# Autodesk Inventor assembly: 6P Sprocket
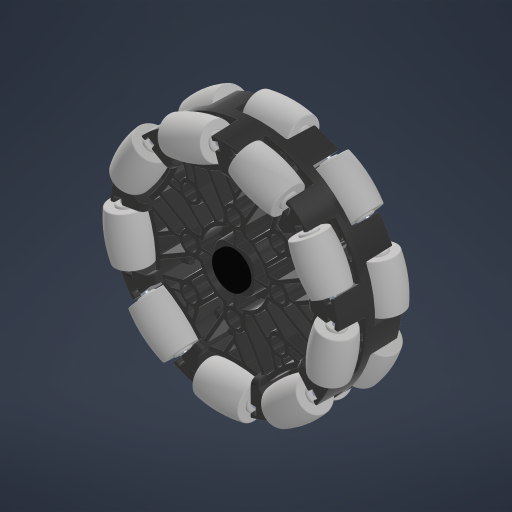
[picture p0: Inventor's stored thumbnail of the model, 512x512]
Saved by Autodesk Inventor 2023.2 (Build 272271000, 271)
## iProperties
Created: 2022-08-02
Part Number: 6P Sprocket
Document SubType Name: Assembly
Designer: ylu12
Author: ylu12
## Documents named in this file (4)
- D:\CAD\Parts\standard\Motion\Wheels\Omni Wheels\Omni Wheel\2.75 Omni AS, Square.iam
- D:\CAD\Parts\standard\Motion\Wheels\Omni Wheels\Reference Parts\2.75 Omni Antistatic.ipt
- D:\CAD\Parts\standard\Motion\Adapters\Insert Square.ipt
- D:\CAD\Parts\standard\Motion\Wheels\Omni Wheels\Omni Wheel.iam
## Components (3 placed, 3 different names)
1. 2.75 Omni Antistatic
2. Square 1 — Mate:17, Flush:10, Flush:11
3. Square 2 — Flush:9, Flush:10, Flush:11, Mate:18, Angle:1
## Relationships (9: Flush 4, Mate 4, Angle 1)
- [Flush]: 2.75 Omni Antistatic
- [Mate]: 2.75 Omni Antistatic
- [Mate]: 2.75 Omni Antistatic
- Flush:9 (6.35 mm): Square 2
- Mate:17 (6.35 mm): Square 1
- Flush:10: Square 1 ↔ Square 2
- Flush:11: Square 1 ↔ Square 2
- Mate:18: Square 2
- Angle:1 (0 deg): Square 2
## Named parameters: HalfWheelWidth = 6.35 mm
